# Autodesk Inventor assembly: 14K_036_010_00_A_ZSB_RIM_04_3D_2016022
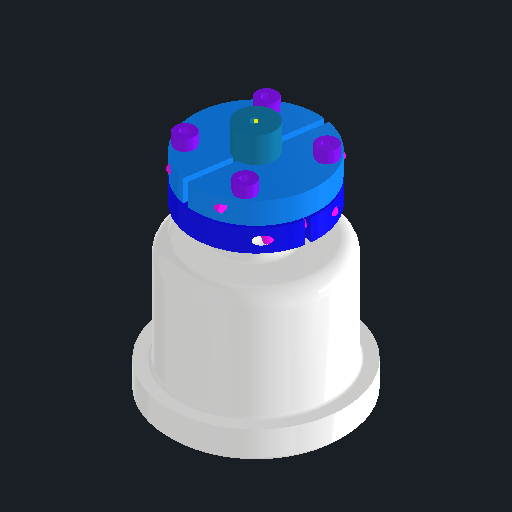
[picture p0: Inventor's stored thumbnail of the model, 512x512]
Saved by Autodesk Inventor 2027 (Build 310192060, 192F)
## iProperties
Created: 2016-03-07
Part Number: 14K_036_010_00_A_ZSB_RIM_04_3D_2016022
Document SubType Name: Assembly
Designer: Halle20
Author: Halle20
## Documents named in this file (5)
- C:\Users\kw\OneDrive\Documents\Uni\Masterthesis\Spezialisierungsmodul\InventorZeichnungen_Konrad\4er-AktuellesDesign\14K_036_010_00_A_ZSB_RIM_04_3D_2016022.iam
- C:\Users\kw\OneDrive\Documents\Uni\Masterthesis\Spezialisierungsmodul\InventorZeichnungen_Konrad\4er-AktuellesDesign\Baugruppe3.iam
- C:\Users\kw\OneDrive\Documents\Uni\Masterthesis\Spezialisierungsmodul\InventorZeichnungen_Konrad\4er-AktuellesDesign\Baugruppe4.iam
- C:\Users\kw\OneDrive\Documents\Uni\Masterthesis\Spezialisierungsmodul\InventorZeichnungen_Konrad\4er-AktuellesDesign\LangmuirProbe_Scetch.ipt
- C:\Users\kw\OneDrive\Documents\Uni\Masterthesis\Spezialisierungsmodul\InventorZeichnungen_Konrad\4er-AktuellesDesign\CatcherModel.ipt
## Components (4 placed, 4 different names)
1. 14K_036_030_40_A_GEFAESS_SPULE_3D.1 [sub-assembly] — Mate:1, Mate:2
2. 14K_036_040_10_A_GASEINLASS_3D.1 [sub-assembly] — Insert:1, Insert:2, Mate:1, Mate:2
3. LangmuirProbe_Scetch:1 — Insert:1
4. CatcherModel:1 — Insert:2
## Relationships (4: Insert 2, Mate 2)
- Insert:1: 14K_036_040_10_A_GASEINLASS_3D.1 ↔ LangmuirProbe_Scetch:1
- Insert:2: 14K_036_040_10_A_GASEINLASS_3D.1 ↔ CatcherModel:1
- Mate:1: 14K_036_030_40_A_GEFAESS_SPULE_3D.1 ↔ 14K_036_040_10_A_GASEINLASS_3D.1
- Mate:2: 14K_036_030_40_A_GEFAESS_SPULE_3D.1 ↔ 14K_036_040_10_A_GASEINLASS_3D.1
